# Autodesk Inventor assembly: Frame V2
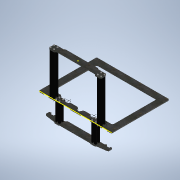
[picture p0: Inventor's stored thumbnail of the model, 180x180]
Saved by Autodesk Inventor 2020.3 (Build 243373010, 373A)
## iProperties
Created: 2019-06-17
Part Number: Frame V2
Document SubType Name: Assembly
Designer: pepd9
Author: pepd9
## Documents named in this file (7)
- D:\Designs\MK3PRO P1\FRAME\Frame V2.iam
- D:\Designs\MK3PRO P1\FRAME\FRONT PLATE P1.2.ipt
- D:\Designs\MK3PRO P1\FRAME\Long Extrusion.ipt
- D:\Designs\MK3PRO P1\COMPONENTS\90128A234_ZNC-PLTD ALLOY STL SCKT HEAD CAP SCREW.ipt
- D:\Designs\MK3PRO P1\FRAME\Short Extrusion.ipt
- D:\Designs\MK3PRO P1\FRAME\REAR PLATE P1.2.ipt
- D:\Designs\MK3PRO P1\FRAME\CENTER FRAME P2.0.ipt
## Components (39 placed, 6 different names)
1. CENTER FRAME P2.0:1 — Mate:1, Mate:2, Mate:3, Mate:4, Mate:5, Mate:6, Mate:7, Mate:8, Mate:9, Flush:1, Mate:23, Mate:24, Mate:25, Mate:28, Mate:37, Mate:38, Mate:39, Mate:40, Mate:41, Mate:42, Mate:43, Mate:44, Mate:45, Mate:46, Mate:47, Mate:48, Mate:49, Mate:50, Mate:51, Mate:52, Mate:53, Mate:54, Mate:55, Mate:56, Mate:57, Mate:58, Mate:59, Mate:60, Mate:61, Mate:62, Mate:63, Mate:64, Mate:65, Mate:66
2. Long Extrusion:1 — Mate:1, Mate:10, Mate:11, Mate:229
3. 90128A234_ZNC-PLTD ALLOY STL SCKT HEAD CAP SCREW:1 — Mate:2, Mate:3, Mate:10
4. 90128A234_ZNC-PLTD ALLOY STL SCKT HEAD CAP SCREW:2 — Mate:6, Mate:7
5. 90128A234_ZNC-PLTD ALLOY STL SCKT HEAD CAP SCREW:3 — Mate:5, Mate:8
6. 90128A234_ZNC-PLTD ALLOY STL SCKT HEAD CAP SCREW:4 — Mate:4, Mate:9, Mate:11
7. 90128A234_ZNC-PLTD ALLOY STL SCKT HEAD CAP SCREW:5 — Mate:231
8. 90128A234_ZNC-PLTD ALLOY STL SCKT HEAD CAP SCREW:6
9. 90128A234_ZNC-PLTD ALLOY STL SCKT HEAD CAP SCREW:7 — Mate:230
10. 90128A234_ZNC-PLTD ALLOY STL SCKT HEAD CAP SCREW:8
11. Long Extrusion:2 — Mate:25, Mate:28
12. 90128A234_ZNC-PLTD ALLOY STL SCKT HEAD CAP SCREW:9
13. 90128A234_ZNC-PLTD ALLOY STL SCKT HEAD CAP SCREW:10
14. 90128A234_ZNC-PLTD ALLOY STL SCKT HEAD CAP SCREW:11
15. 90128A234_ZNC-PLTD ALLOY STL SCKT HEAD CAP SCREW:12
16. 90128A234_ZNC-PLTD ALLOY STL SCKT HEAD CAP SCREW:13 — Mate:37, Mate:44
17. 90128A234_ZNC-PLTD ALLOY STL SCKT HEAD CAP SCREW:14 — Mate:38, Mate:42
18. 90128A234_ZNC-PLTD ALLOY STL SCKT HEAD CAP SCREW:15 — Mate:39, Mate:43
19. 90128A234_ZNC-PLTD ALLOY STL SCKT HEAD CAP SCREW:16 — Mate:40, Mate:41
20. Short Extrusion:1 — Mate:45, Mate:46, Mate:47
21. Short Extrusion:2 — Mate:48, Mate:49, Mate:50, Mate:67, Mate:68, Mate:69
22. 90128A234_ZNC-PLTD ALLOY STL SCKT HEAD CAP SCREW:17 — Mate:53, Mate:56
23. 90128A234_ZNC-PLTD ALLOY STL SCKT HEAD CAP SCREW:18 — Mate:54, Mate:58
24. 90128A234_ZNC-PLTD ALLOY STL SCKT HEAD CAP SCREW:19 — Mate:51, Mate:55
25. 90128A234_ZNC-PLTD ALLOY STL SCKT HEAD CAP SCREW:20 — Mate:52, Mate:57
26. 90128A234_ZNC-PLTD ALLOY STL SCKT HEAD CAP SCREW:21 — Mate:59, Mate:63
27. 90128A234_ZNC-PLTD ALLOY STL SCKT HEAD CAP SCREW:22 — Mate:60, Mate:64
28. 90128A234_ZNC-PLTD ALLOY STL SCKT HEAD CAP SCREW:23 — Mate:61, Mate:65
29. 90128A234_ZNC-PLTD ALLOY STL SCKT HEAD CAP SCREW:24 — Mate:62, Mate:66
30. REAR PLATE P1.2:1 — Mate:67, Mate:68, Mate:69, Mate:70, Mate:71, Mate:72, Mate:73, Mate:74, Mate:75, Mate:76, Mate:77, Mate:78, Mate:79, Mate:80, Mate:81, Mate:82, Mate:83, Mate:84, Mate:95
31. 90128A234_ZNC-PLTD ALLOY STL SCKT HEAD CAP SCREW:25 — Mate:70, Mate:83
32. 90128A234_ZNC-PLTD ALLOY STL SCKT HEAD CAP SCREW:26 — Mate:71, Mate:81
33. 90128A234_ZNC-PLTD ALLOY STL SCKT HEAD CAP SCREW:27 — Mate:73, Mate:84
34. 90128A234_ZNC-PLTD ALLOY STL SCKT HEAD CAP SCREW:28 — Mate:72, Mate:82
35. 90128A234_ZNC-PLTD ALLOY STL SCKT HEAD CAP SCREW:29 — Mate:76, Mate:78
36. 90128A234_ZNC-PLTD ALLOY STL SCKT HEAD CAP SCREW:30 — Mate:74, Mate:77
37. 90128A234_ZNC-PLTD ALLOY STL SCKT HEAD CAP SCREW:31 — Mate:75, Mate:79
38. 90128A234_ZNC-PLTD ALLOY STL SCKT HEAD CAP SCREW:32 — Mate:80, Mate:95
39. FRONT PLATE P1.2:1 — Mate:229, Mate:230, Mate:231
## Relationships (68: Mate 67, Flush 1)
- Mate:1: CENTER FRAME P2.0:1 ↔ Long Extrusion:1
- Mate:2: CENTER FRAME P2.0:1 ↔ 90128A234_ZNC-PLTD ALLOY STL SCKT HEAD CAP SCREW:1
- Mate:3: CENTER FRAME P2.0:1 ↔ 90128A234_ZNC-PLTD ALLOY STL SCKT HEAD CAP SCREW:1
- Mate:4: CENTER FRAME P2.0:1 ↔ 90128A234_ZNC-PLTD ALLOY STL SCKT HEAD CAP SCREW:4
- Mate:5: CENTER FRAME P2.0:1 ↔ 90128A234_ZNC-PLTD ALLOY STL SCKT HEAD CAP SCREW:3
- Mate:6: CENTER FRAME P2.0:1 ↔ 90128A234_ZNC-PLTD ALLOY STL SCKT HEAD CAP SCREW:2
- Mate:7: CENTER FRAME P2.0:1 ↔ 90128A234_ZNC-PLTD ALLOY STL SCKT HEAD CAP SCREW:2
- Mate:8: CENTER FRAME P2.0:1 ↔ 90128A234_ZNC-PLTD ALLOY STL SCKT HEAD CAP SCREW:3
- Mate:9: CENTER FRAME P2.0:1 ↔ 90128A234_ZNC-PLTD ALLOY STL SCKT HEAD CAP SCREW:4
- Mate:10: Long Extrusion:1 ↔ 90128A234_ZNC-PLTD ALLOY STL SCKT HEAD CAP SCREW:1
- Mate:11: Long Extrusion:1 ↔ 90128A234_ZNC-PLTD ALLOY STL SCKT HEAD CAP SCREW:4
- Flush:1 (-245 mm): CENTER FRAME P2.0:1
- Mate:23: CENTER FRAME P2.0:1
- Mate:24 (-24.5 mm): CENTER FRAME P2.0:1
- Mate:25: CENTER FRAME P2.0:1 ↔ Long Extrusion:2
- Mate:28: CENTER FRAME P2.0:1 ↔ Long Extrusion:2
- Mate:37: CENTER FRAME P2.0:1 ↔ 90128A234_ZNC-PLTD ALLOY STL SCKT HEAD CAP SCREW:13
- Mate:38: CENTER FRAME P2.0:1 ↔ 90128A234_ZNC-PLTD ALLOY STL SCKT HEAD CAP SCREW:14
- Mate:39: CENTER FRAME P2.0:1 ↔ 90128A234_ZNC-PLTD ALLOY STL SCKT HEAD CAP SCREW:15
- Mate:40: CENTER FRAME P2.0:1 ↔ 90128A234_ZNC-PLTD ALLOY STL SCKT HEAD CAP SCREW:16
- Mate:41: CENTER FRAME P2.0:1 ↔ 90128A234_ZNC-PLTD ALLOY STL SCKT HEAD CAP SCREW:16
- Mate:42: CENTER FRAME P2.0:1 ↔ 90128A234_ZNC-PLTD ALLOY STL SCKT HEAD CAP SCREW:14
- Mate:43: CENTER FRAME P2.0:1 ↔ 90128A234_ZNC-PLTD ALLOY STL SCKT HEAD CAP SCREW:15
- Mate:44: CENTER FRAME P2.0:1 ↔ 90128A234_ZNC-PLTD ALLOY STL SCKT HEAD CAP SCREW:13
- Mate:45: CENTER FRAME P2.0:1 ↔ Short Extrusion:1
- Mate:46: CENTER FRAME P2.0:1 ↔ Short Extrusion:1
- Mate:47: CENTER FRAME P2.0:1 ↔ Short Extrusion:1
- Mate:48: CENTER FRAME P2.0:1 ↔ Short Extrusion:2
- Mate:49: CENTER FRAME P2.0:1 ↔ Short Extrusion:2
- Mate:50: CENTER FRAME P2.0:1 ↔ Short Extrusion:2
- Mate:51: CENTER FRAME P2.0:1 ↔ 90128A234_ZNC-PLTD ALLOY STL SCKT HEAD CAP SCREW:19
- Mate:52: CENTER FRAME P2.0:1 ↔ 90128A234_ZNC-PLTD ALLOY STL SCKT HEAD CAP SCREW:20
- Mate:53: CENTER FRAME P2.0:1 ↔ 90128A234_ZNC-PLTD ALLOY STL SCKT HEAD CAP SCREW:17
- Mate:54: CENTER FRAME P2.0:1 ↔ 90128A234_ZNC-PLTD ALLOY STL SCKT HEAD CAP SCREW:18
- Mate:55: CENTER FRAME P2.0:1 ↔ 90128A234_ZNC-PLTD ALLOY STL SCKT HEAD CAP SCREW:19
- Mate:56: CENTER FRAME P2.0:1 ↔ 90128A234_ZNC-PLTD ALLOY STL SCKT HEAD CAP SCREW:17
- Mate:57: CENTER FRAME P2.0:1 ↔ 90128A234_ZNC-PLTD ALLOY STL SCKT HEAD CAP SCREW:20
- Mate:58: CENTER FRAME P2.0:1 ↔ 90128A234_ZNC-PLTD ALLOY STL SCKT HEAD CAP SCREW:18
- Mate:59: CENTER FRAME P2.0:1 ↔ 90128A234_ZNC-PLTD ALLOY STL SCKT HEAD CAP SCREW:21
- Mate:60: CENTER FRAME P2.0:1 ↔ 90128A234_ZNC-PLTD ALLOY STL SCKT HEAD CAP SCREW:22
- Mate:61: CENTER FRAME P2.0:1 ↔ 90128A234_ZNC-PLTD ALLOY STL SCKT HEAD CAP SCREW:23
- Mate:62: CENTER FRAME P2.0:1 ↔ 90128A234_ZNC-PLTD ALLOY STL SCKT HEAD CAP SCREW:24
- Mate:63: CENTER FRAME P2.0:1 ↔ 90128A234_ZNC-PLTD ALLOY STL SCKT HEAD CAP SCREW:21
- Mate:64: CENTER FRAME P2.0:1 ↔ 90128A234_ZNC-PLTD ALLOY STL SCKT HEAD CAP SCREW:22
- Mate:65: CENTER FRAME P2.0:1 ↔ 90128A234_ZNC-PLTD ALLOY STL SCKT HEAD CAP SCREW:23
- Mate:66: CENTER FRAME P2.0:1 ↔ 90128A234_ZNC-PLTD ALLOY STL SCKT HEAD CAP SCREW:24
- Mate:67: Short Extrusion:2 ↔ REAR PLATE P1.2:1
- Mate:68: Short Extrusion:2 ↔ REAR PLATE P1.2:1
- Mate:69: Short Extrusion:2 ↔ REAR PLATE P1.2:1
- Mate:70: REAR PLATE P1.2:1 ↔ 90128A234_ZNC-PLTD ALLOY STL SCKT HEAD CAP SCREW:25
- Mate:71: REAR PLATE P1.2:1 ↔ 90128A234_ZNC-PLTD ALLOY STL SCKT HEAD CAP SCREW:26
- Mate:72: REAR PLATE P1.2:1 ↔ 90128A234_ZNC-PLTD ALLOY STL SCKT HEAD CAP SCREW:28
- Mate:73: REAR PLATE P1.2:1 ↔ 90128A234_ZNC-PLTD ALLOY STL SCKT HEAD CAP SCREW:27
- Mate:74: REAR PLATE P1.2:1 ↔ 90128A234_ZNC-PLTD ALLOY STL SCKT HEAD CAP SCREW:30
- Mate:75: REAR PLATE P1.2:1 ↔ 90128A234_ZNC-PLTD ALLOY STL SCKT HEAD CAP SCREW:31
- Mate:76: REAR PLATE P1.2:1 ↔ 90128A234_ZNC-PLTD ALLOY STL SCKT HEAD CAP SCREW:29
- Mate:77: REAR PLATE P1.2:1 ↔ 90128A234_ZNC-PLTD ALLOY STL SCKT HEAD CAP SCREW:30
- Mate:78: REAR PLATE P1.2:1 ↔ 90128A234_ZNC-PLTD ALLOY STL SCKT HEAD CAP SCREW:29
- Mate:79: REAR PLATE P1.2:1 ↔ 90128A234_ZNC-PLTD ALLOY STL SCKT HEAD CAP SCREW:31
- Mate:80: REAR PLATE P1.2:1 ↔ 90128A234_ZNC-PLTD ALLOY STL SCKT HEAD CAP SCREW:32
- Mate:81: REAR PLATE P1.2:1 ↔ 90128A234_ZNC-PLTD ALLOY STL SCKT HEAD CAP SCREW:26
- Mate:82: REAR PLATE P1.2:1 ↔ 90128A234_ZNC-PLTD ALLOY STL SCKT HEAD CAP SCREW:28
- Mate:83: REAR PLATE P1.2:1 ↔ 90128A234_ZNC-PLTD ALLOY STL SCKT HEAD CAP SCREW:25
- Mate:84: REAR PLATE P1.2:1 ↔ 90128A234_ZNC-PLTD ALLOY STL SCKT HEAD CAP SCREW:27
- Mate:95: REAR PLATE P1.2:1 ↔ 90128A234_ZNC-PLTD ALLOY STL SCKT HEAD CAP SCREW:32
- Mate:229: Long Extrusion:1 ↔ FRONT PLATE P1.2:1
- Mate:230: 90128A234_ZNC-PLTD ALLOY STL SCKT HEAD CAP SCREW:7 ↔ FRONT PLATE P1.2:1
- Mate:231: 90128A234_ZNC-PLTD ALLOY STL SCKT HEAD CAP SCREW:5 ↔ FRONT PLATE P1.2:1
